# Autodesk Inventor assembly: mg996r_2_servo_bottom_middle
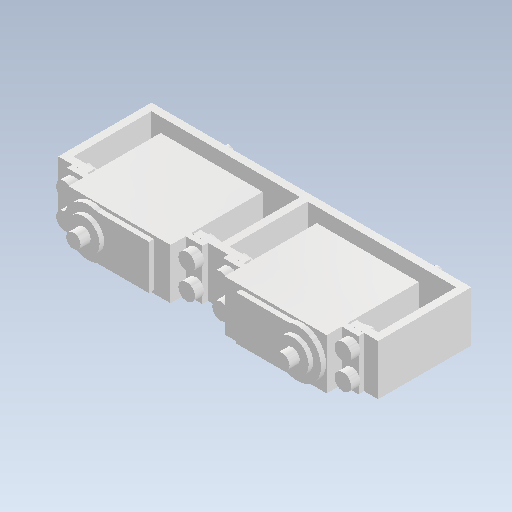
[picture p0: Inventor's stored thumbnail of the model, 512x512]
Saved by Autodesk Inventor 2021.4 (Build 254397000, 397)
## iProperties
Created: 2022-07-24
Part Number: mg996r_2_servo_bottom_middle
Document SubType Name: Assembly
Designer: isamu
Author: isamu
## Documents named in this file (3)
- D:\personal_projects\robot\inventor\2021_matlab_compat _v2\motor_with_frames\mg996r_two_servo_bottom_middle.iam
- D:\personal_projects\robot\inventor\2021_matlab_compat _v2\servo_frames\two_servo_frame_with_nuts.iam
- D:\personal_projects\robot\inventor\2021_matlab_compat _v2\motor\mg996r_motor_with_screws.iam
## Components (3 placed, 2 different names)
1. two_servo_frame_with_nuts:1 [sub-assembly] — Mate:1, Mate:2, Mate:3, Mate:4, Mate:5, Mate:6
2. mg996r_motor_with_screws:1 [sub-assembly] — Mate:4, Mate:5, Mate:6
3. mg996r_motor_with_screws:2 [sub-assembly] — Mate:1, Mate:2, Mate:3
## Relationships (6: Mate 6)
- Mate:1: two_servo_frame_with_nuts:1 ↔ mg996r_motor_with_screws:2
- Mate:2: two_servo_frame_with_nuts:1 ↔ mg996r_motor_with_screws:2
- Mate:3: two_servo_frame_with_nuts:1 ↔ mg996r_motor_with_screws:2
- Mate:4: two_servo_frame_with_nuts:1 ↔ mg996r_motor_with_screws:1
- Mate:5: two_servo_frame_with_nuts:1 ↔ mg996r_motor_with_screws:1
- Mate:6: two_servo_frame_with_nuts:1 ↔ mg996r_motor_with_screws:1
